# Autodesk Inventor assembly: 20_POL_Insert_Linear_Polarizer_spaces
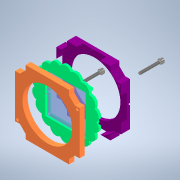
[picture p0: Inventor's stored thumbnail of the model, 180x180]
Saved by Autodesk Inventor 2022 (Build 260153000, 153)
## iProperties
Created: 2021-05-26
Part Number: 20_POL_Insert_Linear_Polarizer_spaces
Document SubType Name: Assembly
Designer: ASUS
Author: ASUS
## Documents named in this file (6)
- C:\Users\ASUS\Desktop\ASP - M.Sc. Photonics\Practical Modules\MODULE 3 - Research Project @IPHT-UC2\7.BUILD_ME\1.build_me_CADs\1. Crossed Polarizers\20_POL_Insert_Linear_Polarizer_spaces.iam
- C:\Users\ASUS\Desktop\ASP - M.Sc. Photonics\Practical Modules\MODULE 3 - Research Project @IPHT-UC2\7.BUILD_ME\1.build_me_CADs\1. Crossed Polarizers\20_POL_Insert_Linear_Polarizer_Guide.ipt
- C:\Users\ASUS\Desktop\ASP - M.Sc. Photonics\Practical Modules\MODULE 3 - Research Project @IPHT-UC2\7.BUILD_ME\1.build_me_CADs\1. Crossed Polarizers\20_POL_Insert_Linear_Polarizer_Lid.ipt
- C:\Users\ASUS\Desktop\ASP - M.Sc. Photonics\Practical Modules\MODULE 3 - Research Project @IPHT-UC2\7.BUILD_ME\1.build_me_CADs\1. Crossed Polarizers\20_POL_Insert_Linear_Polarizer_Wheel.ipt
- C:\Users\ASUS\Desktop\ASP - M.Sc. Photonics\Practical Modules\MODULE 3 - Research Project @IPHT-UC2\7.BUILD_ME\1.build_me_CADs\1. Crossed Polarizers\20_POL_Insert_Linear_Polarizer_Filter.ipt
- C:\Users\ASUS\Documents\Inventor\Content Center Files\R2022\en-US\DIN 912\DIN 912 - M2 x 0,4 x 16 x 15.ipt
## Components (6 placed, 5 different names)
1. 20_POL_Insert_Linear_Polarizer_Guide:1 — Rotational:1
2. 20_POL_Insert_Linear_Polarizer_Lid:1 — Rotational:2, Rotational:3, Rotational:4
3. 20_POL_Insert_Linear_Polarizer_Wheel:1 — Rotational:1, Rotational:2, Rigid:1, Mate:1, Mate:2
4. 20_POL_Insert_Linear_Polarizer_Filter:1 — Rigid:1, Mate:1, Mate:2
5. DIN 912 - replaced by DIN EN ISO 4762 M2 x 16:1 — Rotational:3
6. DIN 912 - replaced by DIN EN ISO 4762 M2 x 16:2 — Rotational:4
## Relationships (7: RevoluteJoint 4, Mate 2, WeldJoint 1)
- Rotational:1 [RevoluteJoint] (-10 mm): 20_POL_Insert_Linear_Polarizer_Guide:1 ↔ 20_POL_Insert_Linear_Polarizer_Wheel:1
- Rotational:2 [RevoluteJoint] (-25 mm): 20_POL_Insert_Linear_Polarizer_Lid:1 ↔ 20_POL_Insert_Linear_Polarizer_Wheel:1
- Rigid:1 [WeldJoint] (-1.5 mm): 20_POL_Insert_Linear_Polarizer_Wheel:1 ↔ 20_POL_Insert_Linear_Polarizer_Filter:1
- Mate:1: 20_POL_Insert_Linear_Polarizer_Wheel:1 ↔ 20_POL_Insert_Linear_Polarizer_Filter:1
- Mate:2: 20_POL_Insert_Linear_Polarizer_Wheel:1 ↔ 20_POL_Insert_Linear_Polarizer_Filter:1
- Rotational:3 [RevoluteJoint] (-25 mm): 20_POL_Insert_Linear_Polarizer_Lid:1 ↔ DIN 912 - replaced by DIN EN ISO 4762 M2 x 16:1
- Rotational:4 [RevoluteJoint] (-25 mm): 20_POL_Insert_Linear_Polarizer_Lid:1 ↔ DIN 912 - replaced by DIN EN ISO 4762 M2 x 16:2
